# Autodesk Inventor assembly: testRoboRescue_Chassis_Frame
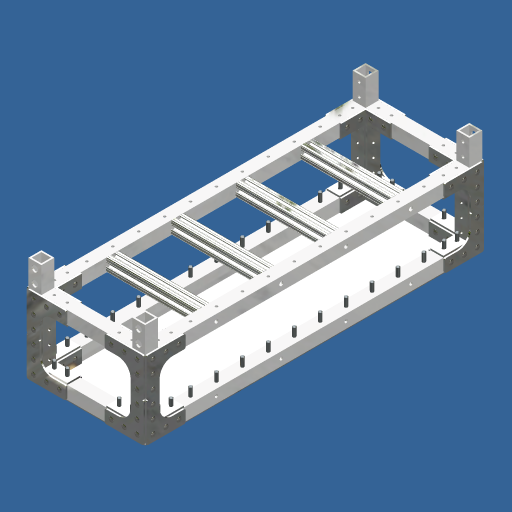
[picture p0: Inventor's stored thumbnail of the model, 512x512]
Saved by Autodesk Inventor 2023 (Build 270158030, 158C)
## iProperties
Created: 2022-03-14
Part Number: testRoboRescue_Chassis_Frame
Document SubType Name: Assembly
Designer: Nebil Oumer
Mass: 5002.95 g
Surface Area: 15217.4 cm^2
Volume: 1975.13 cm^3
Density: 2.53297 g/cm^3
Author: Nebil Oumer
## Documents named in this file (14)
- C:\Users\kumpu\Documents\SBU\CAD\SBRT\Robocup Rescue\Chassis\Frame\Centerpiece\Centerpiece_Frame.iam
- Centerpiece_Frame.iam
- C:\Users\kumpu\Documents\SBU\CAD\SBRT\Robocup Rescue\Chassis\Frame\Centerpiece\Centerpiece_parts\Centerpiece_Frame_heightBar.ipt
- C:\Users\kumpu\Documents\SBU\CAD\SBRT\Robocup Rescue\Chassis\Frame\Centerpiece\Centerpiece_parts\Centerpiece_Frame_widthBar.ipt
- C:\Users\kumpu\Documents\SBU\CAD\SBRT\Robocup Rescue\Chassis\Frame\Centerpiece\Centerpiece_parts\Centerpiece_Frame_lengthBar.ipt
- C:\Users\kumpu\Documents\SBU\CAD\SBRT\Robocup Rescue\Chassis\Frame\Centerpiece\Centerpiece_parts\Centerpiece_bottomPlate.ipt
- C:\Users\kumpu\Documents\SBU\CAD\SBRT\Robocup Rescue\Chassis\Frame\Centerpiece\Centerpiece_parts\Centerpiece_90CornerBracket.ipt
- C:\Users\kumpu\Documents\SBU\CAD\SBRT\Robocup Rescue\Chassis\Frame\Centerpiece\Centerpiece_parts\Centerpiece_FlatGusset.ipt
- C:\Users\kumpu\Documents\SBU\CAD\SBRT\Robocup Rescue\Chassis\Frame\Centerpiece\Centerpiece_parts\Rivet.ipt
- C:\Users\kumpu\Documents\SBU\CAD\SBRT\Robocup Rescue\Chassis\Frame\Centerpiece\Centerpiece_parts\Centerpiece_GussetBolt.ipt
- C:\Users\kumpu\Documents\SBU\CAD\SBRT\Robocup Rescue\Chassis\Frame\Centerpiece\Centerpiece_parts\Centerpiece_GussetBolt_MIR.ipt
- C:\Users\kumpu\Documents\SBU\CAD\SBRT\Robocup Rescue\Chassis\Frame\Centerpiece\Centerpiece_parts\Centerpiece_Frame_BottomLengthBar.ipt
- C:\Users\kumpu\Documents\SBU\CAD\SBRT\Robocup Rescue\Chassis\Frame\Centerpiece\Centerpiece_parts\Centerpiece_Frame_BottomWidthBar.ipt
- C:\Users\kumpu\Documents\SBU\CAD\SBRT\Robocup Rescue\Chassis\Frame\Centerpiece\Centerpiece_parts\T-Slotted Framing.ipt
## Components (205 placed, 12 different names)
1. Centerpiece_bottomPlate:1 — Mate:118, Mate:119, Mate:120, Mate:122, Mate:124, Mate:126, Mate:128, Mate:131, Mate:134, Mate:137
2. Centerpiece_GussetBolt_MIR:1
3. Centerpiece_GussetBolt_MIR:2
4. Centerpiece_GussetBolt_MIR:3
5. Centerpiece_GussetBolt_MIR:4
6. Centerpiece_GussetBolt_MIR:5
7. Centerpiece_GussetBolt_MIR:6
8. Centerpiece_GussetBolt_MIR:7
9. Centerpiece_GussetBolt_MIR:8
10. Centerpiece_Frame_heightBar:1 — Flush:36, Mate:18, Mate:25, Flush:51, Mate:26, Flush:52, Mate:27, Flush:55, Mate:28, Flush:74, Mate:43, Flush:75, Mate:58, Flush:81, Mate:59
11. Centerpiece_Frame_heightBar:2 — Flush:38, Flush:40, Flush:58, Mate:30, Flush:61, Mate:31, Flush:62, Mate:32, Flush:65, Mate:42, Mate:84, Mate:85, Flush:91, Mate:133
12. Centerpiece_Frame_heightBar:3 — Flush:31, Mate:19, Flush:41, Mate:21, Flush:42, Mate:22, Flush:44, Mate:23, Flush:46, Mate:24, Flush:48, Mate:41, Mate:67, Flush:83, Mate:68, Mate:69, Mate:127, Mate:136, Mate:139
13. Centerpiece_Frame_heightBar:4 — Mate:17, Flush:34, Mate:33, Flush:67, Mate:34, Mate:35, Flush:69, Mate:36, Flush:71, Mate:45, Flush:77, Mate:130
14. Centerpiece_Frame_BottomWidthBar:2 — Mate:136, Mate:137, Mate:138
15. Centerpiece_Frame_BottomWidthBar:1 — Mate:133, Mate:134, Mate:135
16. Centerpiece_Frame_widthBar:3 — Flush:8, Flush:40, Mate:29, Flush:59, Mate:43, Flush:75, Mate:80, Mate:81, Flush:89, Mate:88, Mate:89, Flush:93, Mate:98, Flush:98, Mate:100, Flush:99
17. Centerpiece_Frame_widthBar:4 — Flush:101, Mate:139, Mate:140, Flush:102, Mate:141, Mate:142
18. Centerpiece_Frame_BottomLengthBar:1 — Mate:127, Mate:128, Mate:129
19. Centerpiece_Frame_BottomLengthBar:2 — Mate:130, Mate:131, Mate:132
20. Centerpiece_Frame_lengthBar:1 — Mate:17, Flush:34, Flush:38, Flush:63, Flush:66, Mate:42, Mate:72, Flush:85, Mate:73, Mate:99, Mate:105, Symmetry:2, Flush:102
21. Centerpiece_Frame_lengthBar:4 — Flush:8, Flush:31, Flush:36, Mate:18, Flush:50, Flush:74, Mate:41, Flush:82, Mate:60, Mate:101, Mate:102, Flush:100, Flush:101
22. Centerpiece_90CornerBracket:2 — Mate:59, Flush:82, Mate:60
23. Centerpiece_90CornerBracket:3 — Mate:58, Flush:81
24. Centerpiece_90CornerBracket:7
25. Centerpiece_90CornerBracket:8
26. Centerpiece_90CornerBracket:9
27. Centerpiece_90CornerBracket:10 — Mate:84, Mate:85, Flush:91
28. Centerpiece_90CornerBracket:11 — Mate:88, Mate:89, Flush:93
29. Centerpiece_90CornerBracket:12
30. Centerpiece_90CornerBracket:13
31. Centerpiece_90CornerBracket:14
32. Centerpiece_90CornerBracket:15
33. Centerpiece_90CornerBracket:16 — Mate:80, Mate:81, Flush:89
34. Centerpiece_90CornerBracket:17
35. Centerpiece_90CornerBracket:18
36. Centerpiece_90CornerBracket:19 — Mate:72, Flush:85, Mate:73
37. Centerpiece_90CornerBracket:20
38. Centerpiece_90CornerBracket:4 — Flush:83, Mate:68, Mate:69
39. Centerpiece_90CornerBracket:1 — Mate:19, Flush:41
40. Centerpiece_90CornerBracket:6 — Mate:67
41. Centerpiece_90CornerBracket:5
42. Centerpiece_90CornerBracket:21 — Mate:102, Flush:100
43. Centerpiece_90CornerBracket:22 — Mate:98, Mate:99, Flush:98
44. Centerpiece_90CornerBracket:23 — Mate:105, Mate:140
45. Centerpiece_90CornerBracket:24 — Mate:100, Mate:101, Flush:99
46. Centerpiece-FlatGusset:1 — Mate:25, Flush:50, Flush:51, Flush:53, Mate:108, Mate:109
47. Centerpiece-FlatGusset:2 — Mate:21, Flush:42, Flush:47, Mate:49, Mate:50, Mate:106, Mate:107
48. Centerpiece-FlatGusset:3 — Mate:23, Flush:46, Flush:47, Mate:51, Mate:52
49. Centerpiece-FlatGusset:4 — Mate:24, Flush:48, Flush:49, Mate:129
50. Centerpiece-FlatGusset:5 — Mate:29, Flush:58, Flush:59
51. Centerpiece-FlatGusset:6 — Mate:34, Flush:72, Mate:45, Flush:77, Mate:132
52. Centerpiece-FlatGusset:7 — Mate:28
53. Centerpiece-FlatGusset:8 — Mate:22, Flush:44, Flush:49, Mate:138
54. Centerpiece-FlatGusset:9 — Mate:27, Flush:55
55. Centerpiece-FlatGusset:10 — Mate:32, Flush:65
56. Centerpiece-FlatGusset:11 — Mate:36, Flush:71, Flush:72
57. Centerpiece-FlatGusset:12 — Mate:31, Flush:62, Flush:63, Mate:55, Mate:56, Mate:112, Mate:113
58. Centerpiece-FlatGusset:13 — Mate:26, Flush:52, Flush:53, Mate:53, Mate:54, Mate:110, Mate:111
59. Centerpiece-FlatGusset:14 — Mate:33, Flush:66, Flush:67, Flush:70
60. Centerpiece-FlatGusset:15 — Mate:30, Flush:61, Mate:135
61. Centerpiece-FlatGusset:16 — Mate:35, Flush:69, Flush:70
62. Centerpiece_GussetBolt:8 — Mate:124
63. Centerpiece_GussetBolt:7 — Mate:126
64. Centerpiece_GussetBolt:9
65. Centerpiece_GussetBolt:10
66. Centerpiece_GussetBolt:6 — Mate:122
67. Centerpiece_GussetBolt:5 — Mate:120
68. Centerpiece_GussetBolt:11
69. Centerpiece_GussetBolt:12
70. Centerpiece_GussetBolt:1 — Mate:118, Mate:119
71. Centerpiece_GussetBolt:13
72. Centerpiece_GussetBolt:14
73. Centerpiece_GussetBolt:15
74. Centerpiece_GussetBolt:16
75. Centerpiece_GussetBolt:17
76. Centerpiece_GussetBolt:18
77. Centerpiece_GussetBolt:19
78. Centerpiece_GussetBolt:20
79. Centerpiece_GussetBolt:21
80. Centerpiece_GussetBolt:22
81. Centerpiece_GussetBolt:23
82. Centerpiece_GussetBolt:24
83. Centerpiece_GussetBolt:25
84. Centerpiece_GussetBolt:26
85. Centerpiece_GussetBolt:27
86. Centerpiece_GussetBolt:28
87. Centerpiece_GussetBolt:29
88. Centerpiece_GussetBolt:30
89. Centerpiece_GussetBolt:31
90. T-Slotted Framing:1 — Mate:141, Mate:142
91. T-Slotted Framing:2
92. T-Slotted Framing:3
93. T-Slotted Framing:4
94. Rivet:1 — Mate:49, Mate:50
95. Rivet:2
96. Rivet:3
97. Rivet:4
98. Rivet:5
99. Rivet:6
100. Rivet:13
101. Rivet:14
102. Rivet:15
103. Rivet:16
104. Rivet:17
105. Rivet:18
106. Rivet:7 — Mate:51, Mate:52
107. Rivet:8
108. Rivet:9
109. Rivet:10
110. Rivet:11
111. Rivet:12
112. Rivet:19
113. Rivet:20
114. Rivet:21
115. Rivet:22
116. Rivet:23
117. Rivet:24
118. Rivet:25 — Mate:53, Mate:54
119. Rivet:27
120. Rivet:28
121. Rivet:29
122. Rivet:30
123. Rivet:31
124. Rivet:32
125. Rivet:33
126. Rivet:34
127. Rivet:35
128. Rivet:36
129. Rivet:37
130. Rivet:26 — Mate:55, Mate:56
131. Rivet:38
132. Rivet:39
133. Rivet:40
134. Rivet:41
135. Rivet:42
136. Rivet:43
137. Rivet:44
138. Rivet:45
139. Rivet:46
140. Rivet:47
141. Rivet:48
142. Rivet:49 — Mate:106, Mate:107
143. Rivet:53
144. Rivet:54
145. Rivet:55
146. Rivet:56
147. Rivet:57
148. Rivet:58
149. Rivet:59
150. Rivet:81
151. Rivet:82
152. Rivet:83
153. Rivet:84
154. Rivet:85
155. Rivet:86
156. Rivet:87
157. Rivet:88
158. Rivet:51 — Mate:110, Mate:111
159. Rivet:74
160. Rivet:75
161. Rivet:76
162. Rivet:77
163. Rivet:78
164. Rivet:79
165. Rivet:80
166. Rivet:89
167. Rivet:90
168. Rivet:91
169. Rivet:92
170. Rivet:93
171. Rivet:94
172. Rivet:95
173. Rivet:96
174. Rivet:50 — Mate:108, Mate:109
175. Rivet:60
176. Rivet:61
177. Rivet:62
178. Rivet:63
179. Rivet:64
180. Rivet:65
181. Rivet:66
182. Rivet:97
183. Rivet:98
184. Rivet:99
185. Rivet:100
186. Rivet:101
187. Rivet:102
188. Rivet:103
189. Rivet:104
190. Rivet:52 — Mate:112, Mate:113
191. Rivet:67
192. Rivet:68
193. Rivet:69
194. Rivet:70
195. Rivet:71
196. Rivet:72
197. Rivet:73
198. Rivet:105
199. Rivet:106
200. Rivet:107
201. Rivet:108
202. Rivet:109
203. Rivet:110
204. Rivet:111
205. Rivet:112
## Component patterns: (2 elements), (2 elements), (2 elements), (2 elements), (2 elements), (2 elements), (2 elements), (2 elements), (2 elements, first: Centerpiece_GussetBolt:8 + Centerpiece_GussetBolt:7), (2 elements, first: Centerpiece_GussetBolt:6 + Centerpiece_GussetBolt:5), (20 elements, first: Centerpiece_GussetBolt:1), (4 elements, first: T-Slotted Framing:1), (6 elements, first: Rivet:1), Component Pattern 1:2 (6 elements), (6 elements, first: Rivet:7), Component Pattern 2:2 (6 elements), (6 elements, first: Rivet:25), Component Pattern 5:2 (6 elements), (6 elements, first: Rivet:26), Component Pattern 7:2 (6 elements), (2 elements), Component Pattern 13:2 (2 elements), (2 elements), Component Pattern 19:2 (2 elements), (2 elements), Component Pattern 15:2 (2 elements), (2 elements), Component Pattern 17:2 (2 elements), (4 elements, first: Rivet:49), Component Pattern 12:2 (4 elements), Component Pattern 12:3 (4 elements), Component Pattern 12:4 (4 elements), (4 elements, first: Rivet:51), Component Pattern 18:2 (4 elements), Component Pattern 18:3 (4 elements), Component Pattern 18:4 (4 elements), (4 elements, first: Rivet:50), Component Pattern 14:2 (4 elements), Component Pattern 14:3 (4 elements), Component Pattern 14:4 (4 elements), (4 elements, first: Rivet:52), Component Pattern 16:2 (4 elements), Component Pattern 16:3 (4 elements), Component Pattern 16:4 (4 elements)
## Relationships (127: Mate 81, Flush 45, Symmetry 1)
- Flush:8: Centerpiece_Frame_widthBar:3 ↔ Centerpiece_Frame_lengthBar:4
- Flush:31: Centerpiece_Frame_heightBar:3 ↔ Centerpiece_Frame_lengthBar:4
- Mate:17: Centerpiece_Frame_heightBar:4 ↔ Centerpiece_Frame_lengthBar:1
- Flush:34: Centerpiece_Frame_heightBar:4 ↔ Centerpiece_Frame_lengthBar:1
- Flush:36: Centerpiece_Frame_heightBar:1 ↔ Centerpiece_Frame_lengthBar:4
- Mate:18: Centerpiece_Frame_heightBar:1 ↔ Centerpiece_Frame_lengthBar:4
- Flush:38: Centerpiece_Frame_heightBar:2 ↔ Centerpiece_Frame_lengthBar:1
- Flush:40: Centerpiece_Frame_heightBar:2 ↔ Centerpiece_Frame_widthBar:3
- Mate:19: Centerpiece_Frame_heightBar:3 ↔ Centerpiece_90CornerBracket:1
- Flush:41: Centerpiece_Frame_heightBar:3 ↔ Centerpiece_90CornerBracket:1
- Mate:21: Centerpiece_Frame_heightBar:3 ↔ Centerpiece-FlatGusset:2
- Flush:42: Centerpiece_Frame_heightBar:3 ↔ Centerpiece-FlatGusset:2
- Mate:22: Centerpiece_Frame_heightBar:3 ↔ Centerpiece-FlatGusset:8
- Flush:44: Centerpiece_Frame_heightBar:3 ↔ Centerpiece-FlatGusset:8
- Mate:23: Centerpiece_Frame_heightBar:3 ↔ Centerpiece-FlatGusset:3
- Flush:46: Centerpiece_Frame_heightBar:3 ↔ Centerpiece-FlatGusset:3
- Flush:47: Centerpiece-FlatGusset:2 ↔ Centerpiece-FlatGusset:3
- Mate:24: Centerpiece_Frame_heightBar:3 ↔ Centerpiece-FlatGusset:4
- Flush:48: Centerpiece_Frame_heightBar:3 ↔ Centerpiece-FlatGusset:4
- Flush:49: Centerpiece-FlatGusset:4 ↔ Centerpiece-FlatGusset:8
- Mate:25: Centerpiece_Frame_heightBar:1 ↔ Centerpiece-FlatGusset:1
- Flush:50: Centerpiece_Frame_lengthBar:4 ↔ Centerpiece-FlatGusset:1
- Flush:51: Centerpiece_Frame_heightBar:1 ↔ Centerpiece-FlatGusset:1
- Mate:26: Centerpiece_Frame_heightBar:1 ↔ Centerpiece-FlatGusset:13
- Flush:52: Centerpiece_Frame_heightBar:1 ↔ Centerpiece-FlatGusset:13
- Flush:53: Centerpiece-FlatGusset:1 ↔ Centerpiece-FlatGusset:13
- Mate:27: Centerpiece_Frame_heightBar:1 ↔ Centerpiece-FlatGusset:9
- Flush:55: Centerpiece_Frame_heightBar:1 ↔ Centerpiece-FlatGusset:9
- Mate:28: Centerpiece_Frame_heightBar:1 ↔ Centerpiece-FlatGusset:7
- Mate:29: Centerpiece_Frame_widthBar:3 ↔ Centerpiece-FlatGusset:5
- Flush:58: Centerpiece_Frame_heightBar:2 ↔ Centerpiece-FlatGusset:5
- Flush:59: Centerpiece_Frame_widthBar:3 ↔ Centerpiece-FlatGusset:5
- Mate:30: Centerpiece_Frame_heightBar:2 ↔ Centerpiece-FlatGusset:15
- Flush:61: Centerpiece_Frame_heightBar:2 ↔ Centerpiece-FlatGusset:15
- Mate:31: Centerpiece_Frame_heightBar:2 ↔ Centerpiece-FlatGusset:12
- Flush:62: Centerpiece_Frame_heightBar:2 ↔ Centerpiece-FlatGusset:12
- Flush:63: Centerpiece_Frame_lengthBar:1 ↔ Centerpiece-FlatGusset:12
- Mate:32: Centerpiece_Frame_heightBar:2 ↔ Centerpiece-FlatGusset:10
- Flush:65: Centerpiece_Frame_heightBar:2 ↔ Centerpiece-FlatGusset:10
- Mate:33: Centerpiece_Frame_heightBar:4 ↔ Centerpiece-FlatGusset:14
- Flush:66: Centerpiece_Frame_lengthBar:1 ↔ Centerpiece-FlatGusset:14
- Flush:67: Centerpiece_Frame_heightBar:4 ↔ Centerpiece-FlatGusset:14
- Mate:34: Centerpiece_Frame_heightBar:4 ↔ Centerpiece-FlatGusset:6
- Mate:35: Centerpiece_Frame_heightBar:4 ↔ Centerpiece-FlatGusset:16
- Flush:69: Centerpiece_Frame_heightBar:4 ↔ Centerpiece-FlatGusset:16
- Flush:70: Centerpiece-FlatGusset:14 ↔ Centerpiece-FlatGusset:16
- Mate:36: Centerpiece_Frame_heightBar:4 ↔ Centerpiece-FlatGusset:11
- Flush:71: Centerpiece_Frame_heightBar:4 ↔ Centerpiece-FlatGusset:11
- Flush:72: Centerpiece-FlatGusset:6 ↔ Centerpiece-FlatGusset:11
- Flush:74 (-50.8 mm): Centerpiece_Frame_heightBar:1 ↔ Centerpiece_Frame_lengthBar:4
- Mate:41: Centerpiece_Frame_heightBar:3 ↔ Centerpiece_Frame_lengthBar:4
- Mate:42: Centerpiece_Frame_heightBar:2 ↔ Centerpiece_Frame_lengthBar:1
- Mate:43: Centerpiece_Frame_heightBar:1 ↔ Centerpiece_Frame_widthBar:3
- Flush:75: Centerpiece_Frame_heightBar:1 ↔ Centerpiece_Frame_widthBar:3
- Mate:45: Centerpiece_Frame_heightBar:4 ↔ Centerpiece-FlatGusset:6
- Flush:77: Centerpiece_Frame_heightBar:4 ↔ Centerpiece-FlatGusset:6
- Mate:49: Centerpiece-FlatGusset:2 ↔ Rivet:1
- Mate:50: Centerpiece-FlatGusset:2 ↔ Rivet:1
- Mate:51: Centerpiece-FlatGusset:3 ↔ Rivet:7
- Mate:52: Centerpiece-FlatGusset:3 ↔ Rivet:7
- Mate:53: Centerpiece-FlatGusset:13 ↔ Rivet:25
- Mate:54: Centerpiece-FlatGusset:13 ↔ Rivet:25
- Mate:55: Centerpiece-FlatGusset:12 ↔ Rivet:26
- Mate:56: Centerpiece-FlatGusset:12 ↔ Rivet:26
- Mate:58: Centerpiece_Frame_heightBar:1 ↔ Centerpiece_90CornerBracket:3
- Flush:81: Centerpiece_Frame_heightBar:1 ↔ Centerpiece_90CornerBracket:3
- Mate:59: Centerpiece_Frame_heightBar:1 ↔ Centerpiece_90CornerBracket:2
- Flush:82: Centerpiece_Frame_lengthBar:4 ↔ Centerpiece_90CornerBracket:2
- Mate:60: Centerpiece_Frame_lengthBar:4 ↔ Centerpiece_90CornerBracket:2
- Mate:67: Centerpiece_Frame_heightBar:3 ↔ Centerpiece_90CornerBracket:6
- Flush:83: Centerpiece_Frame_heightBar:3 ↔ Centerpiece_90CornerBracket:4
- Mate:68: Centerpiece_Frame_heightBar:3 ↔ Centerpiece_90CornerBracket:4
- Mate:69: Centerpiece_Frame_heightBar:3 ↔ Centerpiece_90CornerBracket:4
- Mate:72: Centerpiece_Frame_lengthBar:1 ↔ Centerpiece_90CornerBracket:19
- Flush:85: Centerpiece_Frame_lengthBar:1 ↔ Centerpiece_90CornerBracket:19
- Mate:73: Centerpiece_Frame_lengthBar:1 ↔ Centerpiece_90CornerBracket:19
- Mate:80: Centerpiece_Frame_widthBar:3 ↔ Centerpiece_90CornerBracket:16
- Mate:81: Centerpiece_Frame_widthBar:3 ↔ Centerpiece_90CornerBracket:16
- Flush:89: Centerpiece_Frame_widthBar:3 ↔ Centerpiece_90CornerBracket:16
- Mate:84: Centerpiece_Frame_heightBar:2 ↔ Centerpiece_90CornerBracket:10
- Mate:85: Centerpiece_Frame_heightBar:2 ↔ Centerpiece_90CornerBracket:10
- Flush:91: Centerpiece_Frame_heightBar:2 ↔ Centerpiece_90CornerBracket:10
- Mate:88: Centerpiece_Frame_widthBar:3 ↔ Centerpiece_90CornerBracket:11
- Mate:89: Centerpiece_Frame_widthBar:3 ↔ Centerpiece_90CornerBracket:11
- Flush:93: Centerpiece_Frame_widthBar:3 ↔ Centerpiece_90CornerBracket:11
- Mate:98: Centerpiece_Frame_widthBar:3 ↔ Centerpiece_90CornerBracket:22
- Mate:99: Centerpiece_Frame_lengthBar:1 ↔ Centerpiece_90CornerBracket:22
- Flush:98: Centerpiece_Frame_widthBar:3 ↔ Centerpiece_90CornerBracket:22
- Mate:100: Centerpiece_Frame_widthBar:3 ↔ Centerpiece_90CornerBracket:24
- Mate:101: Centerpiece_Frame_lengthBar:4 ↔ Centerpiece_90CornerBracket:24
- Flush:99: Centerpiece_Frame_widthBar:3 ↔ Centerpiece_90CornerBracket:24
- Mate:102: Centerpiece_Frame_lengthBar:4 ↔ Centerpiece_90CornerBracket:21
- Flush:100: Centerpiece_Frame_lengthBar:4 ↔ Centerpiece_90CornerBracket:21
- Mate:105: Centerpiece_Frame_lengthBar:1 ↔ Centerpiece_90CornerBracket:23
- Mate:106: Centerpiece-FlatGusset:2 ↔ Rivet:49
- Mate:107: Centerpiece-FlatGusset:2 ↔ Rivet:49
- Mate:108: Centerpiece-FlatGusset:1 ↔ Rivet:50
- Mate:109: Centerpiece-FlatGusset:1 ↔ Rivet:50
- Mate:110: Centerpiece-FlatGusset:13 ↔ Rivet:51
- Mate:111: Centerpiece-FlatGusset:13 ↔ Rivet:51
- Mate:112: Centerpiece-FlatGusset:12 ↔ Rivet:52
- Mate:113: Centerpiece-FlatGusset:12 ↔ Rivet:52
- Mate:118: Centerpiece_bottomPlate:1 ↔ Centerpiece_GussetBolt:1
- Mate:119: Centerpiece_bottomPlate:1 ↔ Centerpiece_GussetBolt:1
- Mate:120: Centerpiece_bottomPlate:1 ↔ Centerpiece_GussetBolt:5
- Mate:122: Centerpiece_bottomPlate:1 ↔ Centerpiece_GussetBolt:6
- Mate:124: Centerpiece_bottomPlate:1 ↔ Centerpiece_GussetBolt:8
- Mate:126: Centerpiece_bottomPlate:1 ↔ Centerpiece_GussetBolt:7
- Symmetry:2: Centerpiece_Frame_lengthBar:1
- Mate:127: Centerpiece_Frame_heightBar:3 ↔ Centerpiece_Frame_BottomLengthBar:1
- Mate:128: Centerpiece_bottomPlate:1 ↔ Centerpiece_Frame_BottomLengthBar:1
- Mate:129: Centerpiece_Frame_BottomLengthBar:1 ↔ Centerpiece-FlatGusset:4
- Mate:130: Centerpiece_Frame_heightBar:4 ↔ Centerpiece_Frame_BottomLengthBar:2
- Mate:131: Centerpiece_bottomPlate:1 ↔ Centerpiece_Frame_BottomLengthBar:2
- Mate:132: Centerpiece_Frame_BottomLengthBar:2 ↔ Centerpiece-FlatGusset:6
- Mate:133: Centerpiece_Frame_heightBar:2 ↔ Centerpiece_Frame_BottomWidthBar:1
- Mate:134: Centerpiece_bottomPlate:1 ↔ Centerpiece_Frame_BottomWidthBar:1
- Mate:135: Centerpiece_Frame_BottomWidthBar:1 ↔ Centerpiece-FlatGusset:15
- Mate:136: Centerpiece_Frame_heightBar:3 ↔ Centerpiece_Frame_BottomWidthBar:2
- Mate:137: Centerpiece_bottomPlate:1 ↔ Centerpiece_Frame_BottomWidthBar:2
- Mate:138: Centerpiece_Frame_BottomWidthBar:2 ↔ Centerpiece-FlatGusset:8
- Flush:101: Centerpiece_Frame_widthBar:4 ↔ Centerpiece_Frame_lengthBar:4
- Mate:139: Centerpiece_Frame_heightBar:3 ↔ Centerpiece_Frame_widthBar:4
- Mate:140: Centerpiece_Frame_widthBar:4 ↔ Centerpiece_90CornerBracket:23
- Flush:102: Centerpiece_Frame_widthBar:4 ↔ Centerpiece_Frame_lengthBar:1
- Mate:141: Centerpiece_Frame_widthBar:4 ↔ T-Slotted Framing:1
- Mate:142: Centerpiece_Frame_widthBar:4 ↔ T-Slotted Framing:1
